# Autodesk Inventor assembly: Assembly7
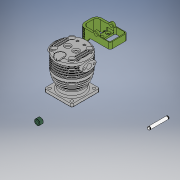
[picture p0: Inventor's stored thumbnail of the model, 180x180]
Saved by Autodesk Inventor 2018 (Build 220112000, 112)
## iProperties
Created: 2023-04-25
Part Number: Assembly7
Document SubType Name: Assembly
Designer: Habib Mohamed
Author: Habib Mohamed
## Documents named in this file (9)
- D:\Inventor\My projects\Rotary Engine\Assembly\Assembly7.iam
- D:\Inventor\My projects\Rotary Engine\Component 13 (Cylinder Liner).ipt
- D:\Inventor\My projects\Rotary Engine\Component 22 (Cylinder Base Gasket).ipt
- D:\Inventor\My projects\Rotary Engine\Component 35(Cylinder Top Gasket).ipt
- D:\Inventor\My projects\Rotary Engine\Component 50(Cylinder Head).ipt
- D:\Inventor\My projects\Rotary Engine\Component 49(Cylinder).ipt
- D:\Inventor\My projects\Rotary Engine\Component 25 (Rocker Arm Axle).ipt
- D:\Inventor\My projects\Rotary Engine\Component 36(Rocker Arm Bracket).ipt
- D:\Inventor\My projects\Rotary Engine\Component 14 (Spacer Sleeve).ipt
## Components (8 placed, 8 different names)
1. Component 13 (Cylinder Liner):1 — Mate:7, Mate:8, Mate:9, Mate:12
2. Component 22 (Cylinder Base Gasket):1 — Mate:11, Mate:12, Mate:13
3. Component 35(Cylinder Top Gasket):1 — Mate:6, Mate:9
4. Component 50(Cylinder Head):1 — Mate:4, Mate:5, Mate:10
5. Component 49(Cylinder):1 — Mate:1, Mate:2, Mate:3, Mate:4, Mate:5, Mate:6, Mate:7, Mate:8, Mate:10, Mate:11, Mate:13
6. Component 25 (Rocker Arm Axle):1
7. Component 36(Rocker Arm Bracket):1
8. Component 14 (Spacer Sleeve):1
## Relationships (13: Mate 13)
- Mate:1: Component 49(Cylinder):1
- Mate:2: Component 49(Cylinder):1
- Mate:3: Component 49(Cylinder):1
- Mate:4: Component 50(Cylinder Head):1 ↔ Component 49(Cylinder):1
- Mate:5: Component 50(Cylinder Head):1 ↔ Component 49(Cylinder):1
- Mate:6: Component 35(Cylinder Top Gasket):1 ↔ Component 49(Cylinder):1
- Mate:7: Component 13 (Cylinder Liner):1 ↔ Component 49(Cylinder):1
- Mate:8: Component 13 (Cylinder Liner):1 ↔ Component 49(Cylinder):1
- Mate:9: Component 13 (Cylinder Liner):1 ↔ Component 35(Cylinder Top Gasket):1
- Mate:10: Component 50(Cylinder Head):1 ↔ Component 49(Cylinder):1
- Mate:11: Component 22 (Cylinder Base Gasket):1 ↔ Component 49(Cylinder):1
- Mate:12: Component 13 (Cylinder Liner):1 ↔ Component 22 (Cylinder Base Gasket):1
- Mate:13: Component 22 (Cylinder Base Gasket):1 ↔ Component 49(Cylinder):1
